# Autodesk Inventor assembly: quad_bai_t_sim
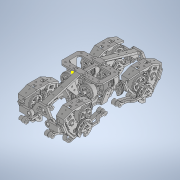
[picture p0: Inventor's stored thumbnail of the model, 180x180]
Saved by Autodesk Inventor 2020 (Build 240168000, 168)
## iProperties
Created: 2021-03-10
Part Number: quad_bai_t_sim
Document SubType Name: Assembly
Designer: Shuang Peng
Author: Shuang Peng
## Documents named in this file (7)
- D:\projects-3\biped_tiny\hardware\sim_mod\quad_bai_t_sim.iam
- D:\projects-3\biped_tiny\hardware\body_shell_1.ipt
- D:\projects-3\biped_tiny\hardware\body_shell_2.ipt
- D:\projects-3\biped_tiny\hardware\sim_mod\reducer_1.iam
- D:\projects-3\biped_tiny\hardware\sim_mod\leg_1_sim.iam
- D:\projects-3\biped_tiny\hardware\sim_mod\leg_1_MIR_sim.iam
- D:\projects-3\biped_tiny\hardware\fr_bearing_s_1.ipt
## Components (12 placed, 6 different names)
1. body_shell_1:1 — Insert:1, Insert:2, Insert:3, Insert:4, Insert:5, Insert:6, Insert:7, Insert:8, Insert:9, Insert:10, Angle:1, Angle:2, Angle:3, Angle:4, Insert:15, Insert:16, Insert:17, Insert:18
2. body_shell_2:1 — Mate:1, Mate:2, Insert:1, Insert:2
3. reducer_1:1 [sub-assembly] — Insert:9, Insert:10, Insert:14
4. reducer_1:2 [sub-assembly] — Insert:7, Insert:8, Insert:11
5. reducer_1:3 [sub-assembly] — Insert:5, Insert:6, Insert:12
6. reducer_1:4 [sub-assembly] — Insert:3, Insert:4, Insert:13
7. leg_1_sim:1 [sub-assembly] — Insert:11, Angle:1
8. leg_1_sim:2 [sub-assembly] — Insert:12, Angle:2
9. leg_1_MIR_sim:1 [sub-assembly] — Insert:14, Angle:4
10. leg_1_MIR_sim:2 [sub-assembly] — Insert:13, Angle:3
11. fr_bearing_s_1:1 — Insert:15, Insert:16
12. fr_bearing_s_1:2 — Insert:17, Insert:18
## Relationships (24: Insert 18, Angle 4, Mate 2)
- Mate:1: body_shell_2:1
- Mate:2: body_shell_2:1
- Insert:1: body_shell_1:1 ↔ body_shell_2:1
- Insert:2: body_shell_1:1 ↔ body_shell_2:1
- Insert:3: body_shell_1:1 ↔ reducer_1:4
- Insert:4: body_shell_1:1 ↔ reducer_1:4
- Insert:5: body_shell_1:1 ↔ reducer_1:3
- Insert:6: body_shell_1:1 ↔ reducer_1:3
- Insert:7: body_shell_1:1 ↔ reducer_1:2
- Insert:8: body_shell_1:1 ↔ reducer_1:2
- Insert:9: body_shell_1:1 ↔ reducer_1:1
- Insert:10: body_shell_1:1 ↔ reducer_1:1
- Insert:11: reducer_1:2 ↔ leg_1_sim:1
- Insert:12: reducer_1:3 ↔ leg_1_sim:2
- Angle:1 (0 deg): body_shell_1:1 ↔ leg_1_sim:1
- Angle:2 (0 deg): body_shell_1:1 ↔ leg_1_sim:2
- Insert:13: reducer_1:4 ↔ leg_1_MIR_sim:2
- Insert:14: reducer_1:1 ↔ leg_1_MIR_sim:1
- Angle:3 (0 deg): body_shell_1:1 ↔ leg_1_MIR_sim:2
- Angle:4 (0 deg): body_shell_1:1 ↔ leg_1_MIR_sim:1
- Insert:15: body_shell_1:1 ↔ fr_bearing_s_1:1
- Insert:16: body_shell_1:1 ↔ fr_bearing_s_1:1
- Insert:17: body_shell_1:1 ↔ fr_bearing_s_1:2
- Insert:18: body_shell_1:1 ↔ fr_bearing_s_1:2
